# Autodesk Inventor assembly: Zusammenbau_DruckLuftMotor
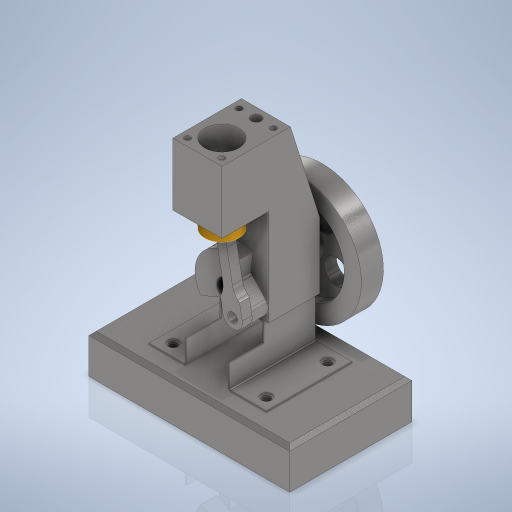
[picture p0: Inventor's stored thumbnail of the model, 512x512]
Saved by Autodesk Inventor 2024 (Build 280153000, 153)
## iProperties
Created: 2024-01-15
Part Number: Zusammenbau_DruckLuftMotor
Document SubType Name: Assembly
Designer: ffogue
Author: ffogue
## Documents named in this file (9)
- C:\Users\ffogue\OneDrive - MuM - OM\Dokumente\Inventor\Motor\Zusammenbau_DruckLuftMotor.iam
- C:\Users\ffogue\OneDrive - MuM - OM\Dokumente\Inventor\Motor\Grundplatte.ipt
- C:\Users\ffogue\OneDrive - MuM - OM\Dokumente\Inventor\Motor\Bügelbefestigung.ipt
- C:\Users\ffogue\OneDrive - MuM - OM\Dokumente\Inventor\Motor\Kolben.ipt
- C:\Users\ffogue\OneDrive - MuM - OM\Dokumente\Inventor\Motor\Pleuel.ipt
- C:\Users\ffogue\OneDrive - MuM - OM\Dokumente\Inventor\Motor\Kurbelzapfen.ipt
- C:\Users\ffogue\OneDrive - MuM - OM\Dokumente\Inventor\Motor\Schwungscheibe.ipt
- C:\Users\ffogue\OneDrive - MuM - OM\Dokumente\Inventor\Motor\Kurbel.ipt
- C:\Users\ffogue\OneDrive - MuM - OM\Dokumente\Inventor\Motor\MotorBlock.ipt
## Components (8 placed, 8 different names)
1. Bügelbefestigung:1 — Einfügen:1, Winkel:1, Einfügen:2, Winkel:2
2. Pleuel:1 — Einfügen:3, Einfügen:7
3. Kurbelzapfen:1 — Einfügen:3, Drehbar:1
4. Kolben:1 — Zylindrisch:1, Drehbar:1
5. MotorBlock:1 — Einfügen:2, Winkel:2, Zylindrisch:1, Einfügen:6, Passend:1
6. Kurbel:1 — Einfügen:7, Winkel:6, Passend:1, Drehung:1
7. Grundplatte:1 — Einfügen:1, Winkel:1
8. Schwungscheibe:1 — Einfügen:6, Motion, Winkel:6, Drehung:1
## Relationships (13: Insert 5, Angle 4, CylindricalJoint 1, RevoluteJoint 1, Mate 1, RelateRotation 1)
- Einfügen:1 [Insert]: Bügelbefestigung:1 ↔ Grundplatte:1
- Winkel:1 [Angle] (270 deg): Bügelbefestigung:1 ↔ Grundplatte:1
- Einfügen:2 [Insert]: Bügelbefestigung:1 ↔ MotorBlock:1
- Winkel:2 [Angle] (0 deg): Bügelbefestigung:1 ↔ MotorBlock:1
- Einfügen:3 [Insert] (-8.8 mm): Pleuel:1 ↔ Kurbelzapfen:1
- Zylindrisch:1 [CylindricalJoint]: Kolben:1 ↔ MotorBlock:1
- Drehbar:1 [RevoluteJoint] (-13.8 mm): Kurbelzapfen:1 ↔ Kolben:1
- Einfügen:6 [Insert] (2 mm): MotorBlock:1 ↔ Schwungscheibe:1
- Motion [Angle] (355 deg): Schwungscheibe:1
- Einfügen:7 [Insert]: Pleuel:1 ↔ Kurbel:1
- Winkel:6 [Angle] (90 deg): Kurbel:1 ↔ Schwungscheibe:1
- Passend:1 [Mate]: MotorBlock:1 ↔ Kurbel:1
- Drehung:1 [RelateRotation] (-1 ul): Kurbel:1 ↔ Schwungscheibe:1
